# Autodesk Inventor assembly: Project Frame
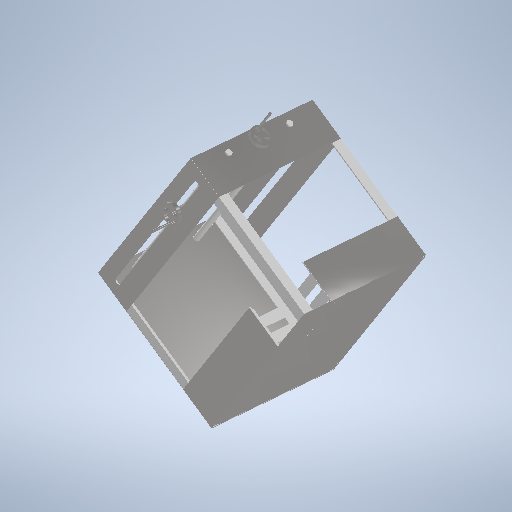
[picture p0: Inventor's stored thumbnail of the model, 512x512]
Saved by Autodesk Inventor 2025.2 (Build 292293000, 293)
## iProperties
Created: 2025-02-04
Part Number: Project Frame
Document SubType Name: Assembly
Designer: Khushal
Author: Khushal
## Documents named in this file (13)
- C:\Users\Khushal\Documents\College\Sem 4\TA212\Project_Latest\Project Frame.iam
- C:\Users\Khushal\Documents\College\Sem 4\TA212\Project_Latest\project base plate.ipt
- C:\Users\Khushal\Documents\College\Sem 4\TA212\Project_Latest\project MS angle.ipt
- C:\Users\Khushal\Documents\College\Sem 4\TA212\Project_Latest\project Backrestfinal.ipt
- C:\Users\Khushal\Documents\College\Sem 4\TA212\Project_Latest\project slot.iam
- C:\Users\Khushal\Documents\College\Sem 4\TA212\Project_Latest\project support plate small.ipt
- C:\Users\Khushal\Documents\College\Sem 4\TA212\Project_Latest\project side supporting plate.ipt
- C:\Users\Khushal\Documents\College\Sem 4\TA212\Project_Latest\project slit.ipt
- C:\Users\Khushal\Documents\College\Sem 4\TA212\Project_Latest\project supporting plate.ipt
- C:\Users\Khushal\Documents\College\Sem 4\TA212\Project_Latest\project front supporting plate.ipt
- C:\Users\Khushal\Documents\College\Sem 4\TA212\Project\leadscrew_modified.ipt
- C:\Users\Khushal\Documents\College\Sem 4\TA212\Project\leadscrew_modified_long.ipt
- C:\Users\Khushal\Documents\College\Sem 4\TA212\Project\support rod.ipt
## Components (17 placed, 12 different names)
1. project base plate:1 — Mate:1, Rigid:1, Mate:2, Mate:3, Mate:4, Rigid:2, Rigid:3, Rigid:4, Mate:11
2. project MS angle:1 — Mate:3, Rigid:3, Mate:8, Mate:13, Rigid:10, Mate:15, Rigid:12, Rigid:14, Rigid:15
3. project MS angle:2 — Mate:1, Rigid:1, Mate:12
4. project MS angle:3 — Mate:4, Rigid:2, Rigid:6, Mate:16, Rigid:13, Rigid:16
5. project MS angle:4 — Mate:2, Rigid:4, Mate:6, Mate:17
6. project Backrestfinal:1 — Mate:6, Rigid:6, Insert:4, Insert:5, Rotational:1
7. project side supporting plate:1 — Mate:8, Mate:9, Rigid:14
8. project slot:1 [sub-assembly] — Mate:9, Mate:11, Mate:18
9. project slit:1 — Mate:12, Rigid:16
10. project support plate small:1 — Mate:13, Rigid:10
11. project supporting plate:2 — Mate:15, Rigid:12
12. project front supporting plate:1 — Mate:16, Rigid:13, Mate:18
13. leadscrew_modified:1
14. leadscrew_modified_long:1 — Rotational:1
15. project slit:2 — Mate:17, Rigid:15
16. support rod:1 — Insert:4
17. support rod:2 — Insert:5
## Relationships (28: Mate 14, WeldJoint 11, Insert 2, RevoluteJoint 1)
- Mate:1: project base plate:1 ↔ project MS angle:2
- Rigid:1 [WeldJoint]: project base plate:1 ↔ project MS angle:2
- Mate:2: project base plate:1 ↔ project MS angle:4
- Mate:3: project base plate:1 ↔ project MS angle:1
- Mate:4: project base plate:1 ↔ project MS angle:3
- Rigid:2 [WeldJoint]: project base plate:1 ↔ project MS angle:3
- Rigid:3 [WeldJoint]: project base plate:1 ↔ project MS angle:1
- Rigid:4 [WeldJoint]: project base plate:1 ↔ project MS angle:4
- Mate:6: project MS angle:4 ↔ project Backrestfinal:1
- Rigid:6 [WeldJoint]: project MS angle:3 ↔ project Backrestfinal:1
- Mate:8: project MS angle:1 ↔ project side supporting plate:1
- Mate:9: project side supporting plate:1 ↔ project slot:1
- Mate:11: project base plate:1 ↔ project slot:1
- Mate:12: project MS angle:2 ↔ project slit:1
- Mate:13: project MS angle:1 ↔ project support plate small:1
- Rigid:10 [WeldJoint]: project MS angle:1 ↔ project support plate small:1
- Mate:15: project MS angle:1 ↔ project supporting plate:2
- Rigid:12 [WeldJoint]: project MS angle:1 ↔ project supporting plate:2
- Mate:16: project MS angle:3 ↔ project front supporting plate:1
- Rigid:13 [WeldJoint]: project MS angle:3 ↔ project front supporting plate:1
- Rigid:14 [WeldJoint]: project MS angle:1 ↔ project side supporting plate:1
- Mate:17: project MS angle:4 ↔ project slit:2
- Rigid:15 [WeldJoint]: project MS angle:1 ↔ project slit:2
- Insert:4 (-5 mm): project Backrestfinal:1 ↔ support rod:1
- Insert:5 (-5 mm): project Backrestfinal:1 ↔ support rod:2
- Mate:18: project slot:1 ↔ project front supporting plate:1
- Rotational:1 [RevoluteJoint] (-5 mm): project Backrestfinal:1 ↔ leadscrew_modified_long:1
- Rigid:16 [WeldJoint]: project MS angle:3 ↔ project slit:1
